(part 1 of 8)
# Autodesk Inventor assembly: Assembly1
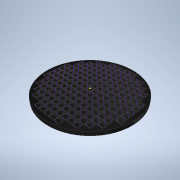
[picture p0: Inventor's stored thumbnail of the model, 180x180]
Saved by Autodesk Inventor 2022 (Build 260153000, 153)
## iProperties
Created: 2022-02-07
Part Number: Assembly1
Document SubType Name: Assembly
Designer: joshw
Author: joshw
## Documents named in this file (5)
- D:\Fab_Labs\Week_3\Inventor_3D\Final_Project_Trial_1\ASSEMBLY\Assembly1.iam
- D:\Fab_Labs\Week_3\Inventor_3D\Final_Project_Trial_1\disk holder.ipt
- D:\Fab_Labs\Week_3\Inventor_3D\Final_Project_Trial_1\coin.ipt
- D:\Fab_Labs\Week_3\Inventor_3D\Final_Project_Trial_1\ASSEMBLY\Coil.ipt
- D:\Fab_Labs\Week_3\Inventor_3D\Final_Project_Trial_1\ASSEMBLY\FRAME.ipt
## Components (710 placed, 4 different names)
1. disk holder:1 — Rotational:1, Angle:1, Mate:3, Mate:4, Angle:2, Mate:5, Angle:3, Mate:10, Mate:14, Mate:15, Mate:16
2. Coil:1 — Mate:3, Mate:4, Angle:2
3. Coil:2 — Mate:5, Angle:3, Mate:10
4. coin:1 — Rotational:1, Angle:1
5. FRAME:1 — Mate:11, Mate:12, Mate:13, Mate:15, Mate:16, Mate:21, Flush:1, Mate:22, Mate:27, Flush:2, Mate:28, Flush:3, Mate:77, Mate:78, Flush:4, Mate:79, Mate:80, Flush:5, Mate:81, Mate:82, Mate:83, Flush:6, Mate:84, Flush:7, Mate:85, Mate:86, Flush:8, Mate:87, Mate:88, Flush:9, Mate:89, Mate:90, Mate:91, Flush:10, Mate:92, Mate:94, Flush:11, Mate:95, Flush:12, Mate:96, Flush:13, Mate:98, Mate:99, Flush:14, Mate:100, Mate:121, Flush:15, Mate:122, Flush:16, Mate:123, Mate:124, Flush:17, Mate:125, Mate:126, Flush:18, Mate:127, Mate:128, Flush:19, Mate:129, Mate:130, Flush:20, Mate:147, Mate:148, Flush:21, Mate:149, Mate:150, Flush:22, Mate:151, Mate:152, Flush:23, Mate:153, Mate:154, Flush:24, Mate:207, Mate:208, Flush:25, Mate:209, Mate:210, Flush:26, Mate:211, Mate:212, Flush:27, Mate:213, Mate:214, Flush:28, Mate:215, Mate:216, Flush:29, Mate:217, Mate:218, Flush:30, Mate:219, Mate:220, Flush:31, Flush:32, Flush:33, Flush:34, Flush:35, Flush:36, Flush:37, Flush:38, Flush:39, Flush:40, Mate:271, Mate:272, Flush:41, Flush:42, Flush:43, Mate:277, Mate:278, Flush:44, Mate:335, Mate:338, Mate:339, Mate:340, Mate:343, Mate:344, Mate:345, Mate:390, Mate:391, Mate:392, Mate:393, Mate:394, Mate:395, Mate:396, Mate:397, Mate:398, Mate:399, Mate:400, Mate:401, Mate:450, Mate:451, Mate:452, Mate:453, Mate:454, Mate:455, Mate:456, Mate:457, Mate:458, Mate:459, Mate:460, Mate:461, Mate:462, Flush:117, Mate:499, Mate:500, Mate:501, Mate:502, Mate:503, Mate:504, Mate:505, Mate:506, Mate:507, Mate:508, Flush:134, Mate:513, Mate:514, Flush:135, Mate:559, Mate:560, Mate:561, Mate:562, Mate:563, Mate:564, Mate:565, Mate:566, Mate:567, Mate:568, Mate:569, Mate:570, Flush:156, Mate:607, Mate:608, Mate:609, Mate:610, Mate:611, Mate:612, Mate:613, Mate:614, Mate:615, Mate:616, Flush:173, Mate:657, Mate:658, Mate:659, Mate:660, Mate:661, Mate:662, Mate:663, Mate:664, Mate:665, Mate:666, Mate:667, Flush:192, Mate:702, Mate:703, Mate:704, Mate:705, Mate:706, Mate:707, Mate:708, Mate:709, Mate:742, Mate:743, Mate:744, Mate:745, Mate:746, Mate:747, Mate:748, Mate:749, Mate:750, Flush:218, Mate:775, Mate:776, Mate:777, Mate:778, Mate:779, Mate:780, Mate:781, Flush:229, Mate:806, Mate:812, Mate:813, Mate:814, Mate:815, Mate:816, Mate:817, Flush:234, Mate:838, Mate:839, Mate:840, Mate:841, Mate:842, Mate:843, Flush:243, Mate:864, Mate:865, Mate:866, Mate:867, Mate:868, Mate:869, Mate:886, Mate:887, Flush:254, Mate:888, Mate:889, Mate:890, Flush:260, Mate:919, Mate:920, Mate:921, Mate:922, Mate:923, Mate:924, Mate:925, Mate:926, Mate:927, Mate:928, Mate:929, Flush:265, Mate:966, Mate:967, Flush:266, Mate:968, Mate:969, Mate:970, Mate:971, Mate:972, Mate:973, Mate:974, Mate:975, Mate:976, Mate:977, Mate:978, Mate:979, Mate:980, Mate:981, Mate:982, Mate:983, Mate:984, Mate:985, Mate:986, Mate:987, Mate:988, Mate:989, Mate:990, Mate:991, Mate:992, Mate:993, Mate:994, Mate:995, Mate:996, Mate:997, Mate:998, Mate:999, Mate:1000, Mate:1001, Mate:1002, Mate:1003, Mate:1004, Mate:1005, Mate:1006, Mate:1007, Mate:1008, Mate:1009, Mate:1010, Mate:1011, Flush:274, Mate:1016, Mate:1017, Mate:1034, Mate:1035, Mate:1036, Mate:1037, Mate:1038
6. disk holder:2 — Mate:21, Flush:1, Mate:22
7. coin:2
8. Coil:3
9. Coil:4
10. disk holder:3 — Mate:27, Flush:2, Mate:28
11. coin:3
12. Coil:5
13. Coil:6
14. disk holder:4 — Flush:3, Mate:77, Mate:78
15. coin:4
16. Coil:7
17. Coil:8
18. disk holder:5 — Mate:91, Flush:10, Mate:92
19. coin:5
20. Coil:9
21. Coil:10
22. disk holder:6 — Flush:9, Mate:89, Mate:90
23. coin:6
24. Coil:11
25. Coil:12
26. disk holder:7 — Flush:8, Mate:87, Mate:88
27. coin:7
28. Coil:13
29. Coil:14
30. disk holder:8 — Flush:4, Mate:79, Mate:80
31. coin:8
32. Coil:15
33. Coil:16
34. disk holder:9 — Flush:5, Mate:81, Mate:82
35. coin:9
36. Coil:17
37. Coil:18
38. disk holder:10 — Mate:83, Flush:6, Mate:84
39. coin:10
40. Coil:19
41. Coil:20
42. disk holder:11 — Flush:7, Mate:85, Mate:86
43. coin:11
44. Coil:21
45. Coil:22
46. disk holder:12 — Mate:95, Flush:12, Mate:96
47. coin:12
48. Coil:23
49. Coil:24
50. disk holder:13 — Mate:94, Flush:11, Mate:997
51. coin:13
52. Coil:25
53. Coil:26
54. disk holder:14 — Mate:99, Flush:14, Mate:100
55. coin:14
56. Coil:27
57. Coil:28
58. disk holder:15 — Flush:13, Mate:98, Mate:996
59. coin:15
60. Coil:29
61. Coil:30
62. disk holder:16 — Flush:18, Mate:127, Mate:128
63. coin:16
64. Coil:31
65. Coil:32
66. disk holder:17 — Flush:16, Mate:123, Mate:124
67. coin:17
68. Coil:33
69. Coil:34
70. disk holder:18 — Mate:121, Flush:15, Mate:122
71. coin:18
72. Coil:35
73. Coil:36
74. disk holder:19 — Flush:17, Mate:125, Mate:126
75. coin:19
76. Coil:37
77. Coil:38
78. disk holder:20 — Flush:19, Mate:129, Mate:130
79. coin:20
80. Coil:39
81. Coil:40
82. disk holder:21 — Flush:23, Mate:153, Mate:154
83. coin:21
84. Coil:41
85. Coil:42
86. disk holder:22 — Flush:22, Mate:151, Mate:152
87. coin:22
88. Coil:43
89. Coil:44
90. disk holder:23 — Flush:20, Mate:147, Mate:148
91. coin:23
92. Coil:45
93. Coil:46
94. disk holder:24 — Flush:21, Mate:149, Mate:150
95. coin:24
96. Coil:47
97. Coil:48
98. disk holder:25 — Flush:30, Mate:219, Mate:220
99. coin:25
100. Coil:49
101. Coil:50
102. disk holder:26 — Flush:35, Mate:1008, Mate:1009
103. coin:26
104. Coil:51
105. Coil:52
106. disk holder:27 — Flush:32, Mate:1004, Mate:1005
107. coin:27
108. Coil:53
109. Coil:54
110. disk holder:28 — Flush:27, Mate:213, Mate:214
111. coin:28
112. Coil:55
113. Coil:56
114. disk holder:29 — Flush:25, Mate:209, Mate:210
115. coin:29
116. Coil:57
117. Coil:58
118. disk holder:30 — Flush:31, Mate:1006, Mate:1007
119. coin:30
120. Coil:59
121. Coil:60
122. disk holder:31 — Flush:29, Mate:217, Mate:218
123. coin:31
124. Coil:61
125. Coil:62
126. disk holder:32 — Flush:24, Mate:207, Mate:208
127. coin:32
128. Coil:63
129. Coil:64
130. disk holder:33 — Flush:26, Mate:211, Mate:212
131. coin:33
132. Coil:65
133. Coil:66
134. disk holder:34 — Flush:28, Mate:215, Mate:216
135. coin:34
136. Coil:67
137. Coil:68
138. disk holder:35 — Flush:33, Mate:1002, Mate:1003
139. coin:35
140. Coil:69
141. Coil:70
142. disk holder:36 — Flush:34, Mate:998, Mate:999
143. coin:36
144. Coil:71
145. Coil:72
146. disk holder:37 — Flush:36, Mate:1000, Mate:1001
147. coin:37
148. Coil:73
149. Coil:74
150. disk holder:38 — Flush:40, Mate:271, Mate:272
151. coin:38
152. Coil:75
153. Coil:76
154. disk holder:39 — Flush:41, Mate:992, Mate:993
155. coin:39
156. Coil:77
157. Coil:78
158. disk holder:40 — Flush:44, Mate:994, Mate:995
159. coin:40
160. Coil:79
161. Coil:80
162. disk holder:41 — Flush:39, Mate:990, Mate:991
163. coin:41
164. Coil:81
165. Coil:82
166. disk holder:42 — Flush:37, Mate:984, Mate:985
167. coin:42
168. Coil:83
169. Coil:84
170. disk holder:43 — Flush:38, Mate:986, Mate:987
171. coin:43
172. Coil:85
173. Coil:86
174. disk holder:44 — Flush:43, Mate:277, Mate:278
175. coin:44
176. Coil:87
177. Coil:88
178. disk holder:45 — Flush:42, Mate:988, Mate:989
179. coin:45
180. Coil:89
181. Coil:90
182. disk holder:46 — Flush:45, Flush:71, Flush:82, Flush:83, Flush:84, Mate:394
183. coin:46
184. Coil:91
185. Coil:92
186. disk holder:47 — Flush:46, Mate:338, Mate:1011
187. coin:47
188. Coil:93
189. Coil:94
190. disk holder:48 — Flush:45, Flush:46, Mate:335, Mate:1010
191. coin:48
192. Coil:95
193. Coil:96
194. disk holder:50 — Flush:49, Flush:62, Mate:345
195. coin:50
196. Coil:99
197. Coil:100
198. disk holder:51 — Flush:49, Flush:61, Mate:340
199. coin:51
200. Coil:101
201. Coil:102
202. disk holder:53 — Flush:60, Mate:343
203. coin:53
204. Coil:105
205. Coil:106
206. disk holder:55 — Flush:59, Flush:61, Flush:62, Mate:339
207. coin:55
208. Coil:109
209. Coil:110
210. disk holder:57 — Flush:59, Flush:60, Mate:344
211. coin:57
212. Coil:113
213. Coil:114
214. disk holder:59 — Flush:73, Flush:74, Flush:94, Flush:97, Flush:114, Mate:460
215. coin:59
216. Coil:117
217. Coil:118
218. disk holder:60 — Flush:74, Flush:75, Flush:76, Flush:77, Flush:84, Flush:92, Mate:395
219. coin:60
220. Coil:119
221. Coil:120
222. disk holder:61 — Flush:71, Flush:72, Flush:82, Flush:85, Mate:393
223. coin:61
224. Coil:121
225. Coil:122
226. disk holder:62 — Flush:75, Flush:79, Flush:83, Mate:397
227. coin:62
228. Coil:123
229. Coil:124
230. disk holder:63 — Flush:77, Flush:78, Flush:88, Mate:399
231. coin:63
232. Coil:125
233. Coil:126
234. disk holder:64 — Flush:72, Flush:73, Flush:86, Flush:90, Flush:91, Mate:400
235. coin:64
236. Coil:127
237. Coil:128
238. disk holder:65 — Flush:79, Flush:80, Flush:85, Mate:396
239. coin:65
240. Coil:129
241. Coil:130
242. disk holder:66 — Flush:78, Flush:86, Mate:401
243. coin:66
244. Coil:131
245. Coil:132
246. disk holder:67 — Flush:80, Flush:81, Flush:88, Flush:90, Flush:92, Mate:398
247. coin:67
248. Coil:133
249. Coil:134
250. disk holder:68 — Flush:76, Flush:89, Mate:392
251. coin:68
252. Coil:135
253. Coil:136
254. disk holder:69 — Flush:81, Flush:89, Flush:91, Mate:390, Mate:391
255. coin:69
256. Coil:137
257. Coil:138
258. disk holder:70 — Flush:97, Mate:450, Mate:454
259. coin:70
260. Coil:139
261. Coil:140
262. disk holder:71 — Flush:98, Flush:110, Flush:111, Mate:461
263. coin:71
264. Coil:141
265. Coil:142
266. disk holder:72 — Flush:96, Flush:99, Flush:113, Flush:114, Mate:455
267. coin:72
268. Coil:143
269. Coil:144
270. Coil:145
271. disk holder:74 — Flush:94, Flush:95, Flush:96, Flush:98, Flush:112, Flush:113, Mate:451
272. coin:74
273. Coil:147
274. Coil:148
275. disk holder:75 — Flush:95, Flush:111, Flush:112, Mate:459
276. coin:75
277. Coil:149
278. Coil:150
279. disk holder:76 — Flush:100, Flush:102, Flush:104, Flush:109, Flush:110, Mate:462
280. coin:76
281. Coil:151
282. Coil:152
283. disk holder:77 — Flush:99, Flush:100, Flush:101, Flush:107, Flush:108, Mate:453
284. coin:77
285. Coil:153
286. Coil:154
287. disk holder:78 — Flush:101, Flush:105, Mate:452
288. coin:78
289. Coil:155
290. Coil:156
291. disk holder:79 — Flush:102, Flush:105, Flush:106, Mate:458
292. coin:79
293. Coil:157
294. Coil:158
295. disk holder:80 — Flush:103, Flush:104, Flush:108, Flush:109, Mate:456
296. coin:80
297. Coil:159
298. Coil:160
299. disk holder:81 — Flush:103, Flush:106, Flush:107, Mate:457
300. coin:81
301. Coil:161
302. Coil:162
303. disk holder:82 — Flush:117, Flush:118, Flush:126, Mate:499, Mate:500
304. coin:82
305. Coil:163
306. Coil:164
307. disk holder:83 — Flush:118, Flush:119, Flush:126, Flush:127, Mate:501
308. coin:83
309. Coil:165
310. Coil:166
311. disk holder:84 — Flush:119, Flush:120, Flush:127, Flush:128, Mate:502
312. coin:84
313. Coil:167
314. Coil:168
315. disk holder:85 — Flush:120, Flush:121, Flush:128, Flush:129, Mate:503
316. coin:85
317. Coil:169
318. Coil:170
319. disk holder:86 — Flush:121, Flush:122, Flush:129, Flush:130, Mate:504
320. coin:86
321. Coil:171
322. Coil:172
323. disk holder:87 — Flush:122, Flush:123, Flush:130, Flush:131, Mate:505
324. coin:87
325. Coil:173
326. Coil:174
327. disk holder:88 — Flush:123, Flush:124, Flush:131, Flush:132, Mate:506
328. coin:88
329. Coil:175
330. Coil:176
331. disk holder:89 — Flush:124, Flush:125, Flush:132, Flush:133, Mate:507
332. coin:89
333. Coil:177
334. Coil:178
335. disk holder:90 — Flush:125, Flush:133, Mate:508
336. coin:90
337. Coil:179
338. Coil:180
339. disk holder:91 — Flush:134, Mate:513, Mate:514
340. coin:91
341. Coil:181
342. Coil:182
343. disk holder:92 — Flush:136, Flush:137, Flush:138, Flush:139, Mate:561
344. coin:92
345. Coil:183
346. Coil:184
347. disk holder:93 — Flush:138, Flush:139, Flush:140, Flush:141, Flush:149, Mate:562
348. coin:93
349. Coil:185
350. Coil:186
351. disk holder:94 — Flush:135, Mate:559, Flush:136, Flush:137, Mate:560
352. coin:94
353. Coil:187
354. Coil:188
355. disk holder:95 — Flush:140, Flush:141, Flush:142, Flush:143, Flush:147, Flush:150, Flush:151, Mate:565
356. coin:95
357. Coil:189
358. Coil:190
359. disk holder:96 — Flush:142, Flush:149, Mate:563
360. coin:96
361. Coil:191
362. Coil:192
363. disk holder:97 — Flush:143, Flush:144, Flush:150, Mate:564
364. coin:97
365. Coil:193
366. Coil:194
367. disk holder:98 — Flush:144, Flush:145, Flush:151, Flush:155, Mate:566
368. coin:98
369. Coil:195
370. Coil:196
371. disk holder:99 — Flush:145, Flush:146, Flush:152, Flush:155, Mate:567
372. coin:99
373. Coil:197
374. Coil:198
375. disk holder:100 — Flush:146, Flush:152, Flush:153, Mate:568
376. coin:100
377. Coil:199
378. Coil:200
379. disk holder:101 — Flush:147, Flush:148, Flush:153, Flush:154, Mate:569
380. coin:101
381. Coil:201
382. Coil:202
383. disk holder:102 — Flush:148, Flush:154, Mate:570
384. coin:102
385. Coil:203
386. Coil:204
387. disk holder:103 — Flush:164, Flush:169, Mate:611
388. coin:103
389. Coil:205
390. Coil:206
391. disk holder:104 — Flush:163, Flush:172, Mate:609
392. coin:104
393. Coil:207
394. Coil:208
395. disk holder:105 — Flush:161, Flush:162, Flush:164, Flush:167, Mate:612
396. coin:105
397. Coil:209
398. Coil:210
399. disk holder:106 — Flush:159, Flush:160, Flush:166, Flush:167, Flush:168, Mate:615
400. coin:106
401. Coil:211
402. Coil:212
403. disk holder:107 — Flush:156, Mate:607, Flush:157, Flush:165, Flush:169, Flush:170, Flush:172, Mate:613
404. coin:107
405. Coil:213
406. Coil:214
407. disk holder:108 — Flush:157, Flush:158, Flush:159, Flush:165, Flush:166, Flush:171, Mate:616
408. coin:108
409. Coil:215
410. Coil:216
411. disk holder:109 — Flush:158, Flush:170, Mate:608
412. coin:109
413. Coil:217
414. Coil:218
415. disk holder:110 — Flush:160, Flush:161, Flush:168, Mate:614
416. coin:110
417. Coil:219
418. Coil:220
419. disk holder:111 — Flush:162, Flush:163, Flush:171, Mate:610
420. coin:111
421. Coil:221
422. Coil:222
423. disk holder:112 — Flush:173, Mate:657, Flush:174, Flush:182, Mate:658
424. coin:112
425. Coil:223
426. Coil:224
427. disk holder:113 — Flush:174, Flush:175, Flush:182, Flush:183, Mate:659
428. coin:113
429. Coil:225
430. Coil:226
431. disk holder:114 — Flush:175, Flush:176, Flush:183, Flush:184, Mate:660
432. coin:114
433. Coil:227
434. Coil:228
435. disk holder:115 — Flush:177, Flush:178, Flush:185, Flush:186, Mate:662
436. coin:115
437. Coil:229
438. Coil:230
439. disk holder:116 — Flush:178, Flush:179, Flush:186, Flush:187, Flush:188, Mate:664
440. coin:116
441. Coil:231
442. Coil:232
443. disk holder:117 — Flush:181, Flush:189, Flush:190, Mate:666, Flush:191
444. coin:117
445. Coil:233
446. Coil:234
447. disk holder:118 — Flush:190, Mate:667, Flush:191
448. coin:118
449. Coil:235
450. Coil:236
451. disk holder:119 — Flush:176, Flush:177, Flush:184, Flush:185, Mate:661
452. coin:119
453. Coil:237
454. Coil:238
455. disk holder:120 — Flush:179, Flush:180, Flush:187, Mate:663
456. coin:120
457. Coil:239
458. Coil:240
459. disk holder:121 — Flush:180, Flush:181, Flush:188, Flush:189, Mate:665
460. coin:121
461. Coil:241
462. Coil:242
463. disk holder:122 — Mate:701, Flush:192, Flush:193, Mate:702, Mate:703
464. coin:122
465. Coil:243
466. Coil:244
467. disk holder:123 — Mate:700, Mate:701, Flush:193, Flush:194, Flush:195, Mate:704
468. coin:123
469. Coil:245
470. Coil:246
471. disk holder:124 — Mate:699, Mate:700, Flush:194, Mate:705
472. coin:124
473. Coil:247
474. Coil:248
475. disk holder:125 — Mate:698, Mate:699, Flush:195, Flush:196, Mate:706
476. coin:125
477. Coil:249
478. Coil:250
479. disk holder:126 — Mate:697, Mate:698, Flush:196, Flush:197, Mate:707
480. coin:126
481. Coil:251
482. Coil:252
483. disk holder:127 — Mate:696, Mate:697, Flush:197, Flush:198, Mate:708
484. coin:127
485. Coil:253
486. Coil:254
487. disk holder:128 — Mate:696, Flush:198, Mate:709
488. coin:128
489. Coil:255
490. Coil:256
491. disk holder:129 — Flush:199, Flush:212, Mate:742, Mate:743
492. coin:129
493. Coil:257
494. Coil:258
495. disk holder:130 — Flush:199, Flush:200, Flush:211, Flush:212, Mate:744
496. coin:130
497. Coil:259
498. Coil:260
499. disk holder:131 — Flush:200, Flush:201, Flush:210, Flush:211, Mate:745
500. coin:131
501. Coil:261
502. Coil:262
503. disk holder:132 — Flush:201, Flush:202, Flush:209, Flush:210, Mate:746
504. coin:132
505. Coil:263
506. Coil:264
507. disk holder:133 — Flush:202, Flush:203, Flush:208, Flush:209, Mate:747
508. coin:133
509. Coil:265
510. Coil:266
511. disk holder:134 — Flush:203, Flush:204, Flush:207, Flush:208, Mate:748
512. coin:134
513. Coil:267
514. Coil:268
515. disk holder:135 — Flush:204, Flush:205, Flush:206, Flush:207, Mate:749
516. coin:135
517. Coil:269
518. Coil:270
519. disk holder:136 — Flush:205, Flush:206, Mate:750
520. coin:136
521. Coil:271
522. Coil:272
523. disk holder:137 — Flush:213, Flush:218, Flush:219, Mate:775, Mate:776
524. coin:137
525. Coil:273
526. Coil:274
527. disk holder:138 — Flush:213, Flush:214, Flush:219, Flush:220, Mate:777
528. coin:138
529. Coil:275
530. Coil:276
531. disk holder:139 — Flush:214, Flush:215, Flush:220, Flush:221, Mate:778
532. coin:139
533. Coil:277
534. Coil:278
535. disk holder:140 — Flush:215, Flush:216, Flush:221, Flush:222, Mate:779
536. coin:140
537. Coil:279
538. Coil:280
539. disk holder:141 — Flush:216, Flush:217, Flush:222, Flush:223, Mate:780
540. coin:141
541. Coil:281
542. Coil:282
543. disk holder:142 — Flush:217, Flush:223, Mate:781
544. coin:142
545. Coil:283
546. Coil:284
547. disk holder:143 — Flush:224, Flush:229, Mate:806, Mate:807, Mate:812
548. coin:143
549. Coil:285
550. Coil:286
551. disk holder:144 — Flush:224, Flush:225, Mate:807, Mate:808, Mate:813
552. coin:144
553. Coil:287
554. Coil:288
555. disk holder:145 — Flush:225, Flush:226, Mate:808, Mate:809, Mate:814
556. coin:145
557. Coil:289
558. Coil:290
559. disk holder:146 — Flush:226, Flush:227, Mate:809, Mate:810, Mate:815
560. coin:146
561. Coil:291
562. Coil:292
563. disk holder:147 — Flush:227, Flush:228, Mate:810, Mate:811, Mate:816
564. coin:147
565. Coil:293
566. Coil:294
567. disk holder:148 — Flush:228, Mate:811, Mate:817
568. coin:148
569. Coil:295
570. Coil:296
571. disk holder:149 — Flush:230, Flush:234, Flush:235, Mate:838, Mate:839
572. coin:149
573. Coil:297
574. Coil:298
575. disk holder:150 — Flush:230, Flush:231, Flush:235, Flush:236, Mate:840
576. coin:150
577. Coil:299
578. Coil:300
579. disk holder:151 — Flush:231, Flush:232, Flush:236, Flush:237, Mate:841
580. coin:151
581. Coil:301
582. Coil:302
583. disk holder:152 — Flush:232, Flush:233, Flush:237, Flush:238, Mate:842
584. coin:152
585. Coil:303
586. Coil:304
587. disk holder:153 — Flush:233, Flush:238, Mate:843
588. coin:153
589. Coil:305
590. Coil:306
591. disk holder:154 — Flush:239, Flush:244, Mate:864
592. coin:154
593. Coil:307
594. Coil:308
595. disk holder:155 — Flush:239, Flush:240, Flush:244, Flush:245, Mate:867
596. coin:155
597. Coil:309
598. Coil:310
599. disk holder:156 — Flush:240, Flush:241, Flush:245, Flush:246, Mate:868
600. coin:156
601. Coil:311
602. Coil:312
603. disk holder:157 — Flush:241, Flush:242, Flush:246, Flush:247, Mate:865, Mate:866
604. coin:157
605. Coil:313
606. Coil:314
607. disk holder:158 — Flush:242, Flush:243, Flush:247, Mate:869
608. coin:158
609. Coil:315